# Autodesk Inventor assembly: CAMINHÃO BETONEIRA
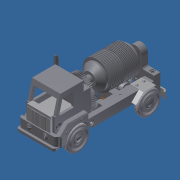
[picture p0: Inventor's stored thumbnail of the model, 180x180]
Saved by Autodesk Inventor 2012 SP2 (Build 160219200, 219)
## iProperties
Created: 2012-07-24
Part Number: CAMINHÃO BETONEIRA
Document SubType Name: Assembly
Designer: bruno.silveira
Author: bruno.silveira
## Documents named in this file (48)
- H:\CAD\BASSOTTI\Documents\DESENHOS.CAD-BRUNOBASSOTTI\DESENHOS-AUTODESK-INVENTOR\CAMINHÃO-BITONEIRA-(SENAI)\CAMINHÃO BETONEIRA.iam
- H:\CAD\BASSOTTI\Documents\DESENHOS.CAD-BRUNOBASSOTTI\DESENHOS-AUTODESK-INVENTOR\CAMINHÃO-BITONEIRA-(SENAI)\MOTOR(3).ipt
- H:\CAD\BASSOTTI\Documents\DESENHOS.CAD-BRUNOBASSOTTI\DESENHOS-AUTODESK-INVENTOR\CAMINHÃO-BITONEIRA-(SENAI)\LAT-CABINE-DIREITA(27).ipt
- H:\CAD\BASSOTTI\Documents\DESENHOS.CAD-BRUNOBASSOTTI\DESENHOS-AUTODESK-INVENTOR\CAMINHÃO-BITONEIRA-(SENAI)\LAT-CABINE-ESQUERDA(28).ipt
- H:\CAD\BASSOTTI\Documents\DESENHOS.CAD-BRUNOBASSOTTI\DESENHOS-AUTODESK-INVENTOR\CAMINHÃO-BITONEIRA-(SENAI)\ISO 2010 - M6x12.ipt
- H:\CAD\BASSOTTI\Documents\DESENHOS.CAD-BRUNOBASSOTTI\DESENHOS-AUTODESK-INVENTOR\CAMINHÃO-BITONEIRA-(SENAI)\PÁRA-LAMAS DIANTEIRO-DIR(1).ipt
- H:\CAD\BASSOTTI\Documents\DESENHOS.CAD-BRUNOBASSOTTI\DESENHOS-AUTODESK-INVENTOR\CAMINHÃO-BITONEIRA-(SENAI)\PÁRA-LAMAS DIANTEIRO-ESQ(1).ipt
- H:\CAD\BASSOTTI\Documents\DESENHOS.CAD-BRUNOBASSOTTI\DESENHOS-AUTODESK-INVENTOR\CAMINHÃO-BITONEIRA-(SENAI)\DIN 661 - A 3 x 16 x 11.ipt
- H:\CAD\BASSOTTI\Documents\DESENHOS.CAD-BRUNOBASSOTTI\DESENHOS-AUTODESK-INVENTOR\CAMINHÃO-BITONEIRA-(SENAI)\TRASEIRA DA CABINE(12).ipt
- H:\CAD\BASSOTTI\Documents\DESENHOS.CAD-BRUNOBASSOTTI\DESENHOS-AUTODESK-INVENTOR\CAMINHÃO-BITONEIRA-(SENAI)\TETO DA CABINE(15).ipt
- H:\CAD\BASSOTTI\Documents\DESENHOS.CAD-BRUNOBASSOTTI\DESENHOS-AUTODESK-INVENTOR\CAMINHÃO-BITONEIRA-(SENAI)\ISO 2010 - M6x10.ipt
- H:\CAD\BASSOTTI\Documents\DESENHOS.CAD-BRUNOBASSOTTI\DESENHOS-AUTODESK-INVENTOR\CAMINHÃO-BITONEIRA-(SENAI)\PÁRA-CHOQUE DIANTEIRO(4).ipt
- H:\CAD\BASSOTTI\Documents\DESENHOS.CAD-BRUNOBASSOTTI\DESENHOS-AUTODESK-INVENTOR\CAMINHÃO-BITONEIRA-(SENAI)\ASSOALHO(8).ipt
- H:\CAD\BASSOTTI\Documents\DESENHOS.CAD-BRUNOBASSOTTI\DESENHOS-AUTODESK-INVENTOR\CAMINHÃO-BITONEIRA-(SENAI)\MANCAL DO EIXO DIANTEIRO(7).ipt
- H:\CAD\BASSOTTI\Documents\DESENHOS.CAD-BRUNOBASSOTTI\DESENHOS-AUTODESK-INVENTOR\CAMINHÃO-BITONEIRA-(SENAI)\ISO 4762 - M6 x 16ISO.ipt
- H:\CAD\BASSOTTI\Documents\DESENHOS.CAD-BRUNOBASSOTTI\DESENHOS-AUTODESK-INVENTOR\CAMINHÃO-BITONEIRA-(SENAI)\EIXO DIANTEIRO(34).ipt
- H:\CAD\BASSOTTI\Documents\DESENHOS.CAD-BRUNOBASSOTTI\DESENHOS-AUTODESK-INVENTOR\CAMINHÃO-BITONEIRA-(SENAI)\RODA(33).ipt
- H:\CAD\BASSOTTI\Documents\DESENHOS.CAD-BRUNOBASSOTTI\DESENHOS-AUTODESK-INVENTOR\CAMINHÃO-BITONEIRA-(SENAI)\ARRUELA ESPECIAL DAS RODAS(31).ipt
- H:\CAD\BASSOTTI\Documents\DESENHOS.CAD-BRUNOBASSOTTI\DESENHOS-AUTODESK-INVENTOR\CAMINHÃO-BITONEIRA-(SENAI)\DIN 913 - M6 x 8.ipt
- H:\CAD\BASSOTTI\Documents\DESENHOS.CAD-BRUNOBASSOTTI\DESENHOS-AUTODESK-INVENTOR\CAMINHÃO-BITONEIRA-(SENAI)\PLACA COM FUROS COORDENADOS(13).ipt
- H:\CAD\BASSOTTI\Documents\DESENHOS.CAD-BRUNOBASSOTTI\DESENHOS-AUTODESK-INVENTOR\CAMINHÃO-BITONEIRA-(SENAI)\CHASSI DIREITO(58).ipt
- H:\CAD\BASSOTTI\Documents\DESENHOS.CAD-BRUNOBASSOTTI\DESENHOS-AUTODESK-INVENTOR\CAMINHÃO-BITONEIRA-(SENAI)\CHASSI ESQUERDO(37).ipt
- H:\CAD\BASSOTTI\Documents\DESENHOS.CAD-BRUNOBASSOTTI\DESENHOS-AUTODESK-INVENTOR\CAMINHÃO-BITONEIRA-(SENAI)\PÁRA-LAMA TRASEIRO(50).ipt
- H:\CAD\BASSOTTI\Documents\DESENHOS.CAD-BRUNOBASSOTTI\DESENHOS-AUTODESK-INVENTOR\CAMINHÃO-BITONEIRA-(SENAI)\Rivet GB_T 827-1986-3 X 12.ipt
- H:\CAD\BASSOTTI\Documents\DESENHOS.CAD-BRUNOBASSOTTI\DESENHOS-AUTODESK-INVENTOR\CAMINHÃO-BITONEIRA-(SENAI)\SUPORTE DO EIXO TRASEIRO(51).ipt
- H:\CAD\BASSOTTI\Documents\DESENHOS.CAD-BRUNOBASSOTTI\DESENHOS-AUTODESK-INVENTOR\CAMINHÃO-BITONEIRA-(SENAI)\EIXO EXCÊNTRICO(53).ipt
- H:\CAD\BASSOTTI\Documents\DESENHOS.CAD-BRUNOBASSOTTI\DESENHOS-AUTODESK-INVENTOR\CAMINHÃO-BITONEIRA-(SENAI)\EIXO DAS ENGRENAGENS(11).ipt
- H:\CAD\BASSOTTI\Documents\DESENHOS.CAD-BRUNOBASSOTTI\DESENHOS-AUTODESK-INVENTOR\CAMINHÃO-BITONEIRA-(SENAI)\BUCHA DA PLACA(38).ipt
- H:\CAD\BASSOTTI\Documents\DESENHOS.CAD-BRUNOBASSOTTI\DESENHOS-AUTODESK-INVENTOR\CAMINHÃO-BITONEIRA-(SENAI)\ENGR.RETA MOTORA(18)\ENGR.RETA MOTORA(18).ipt
- H:\CAD\BASSOTTI\Documents\DESENHOS.CAD-BRUNOBASSOTTI\DESENHOS-AUTODESK-INVENTOR\CAMINHÃO-BITONEIRA-(SENAI)\ENGR.HELICOIDAL MOVIDA(59)\ENGR.HELICOIDAL MOVIDA(59).iam
- H:\CAD\BASSOTTI\Documents\DESENHOS.CAD-BRUNOBASSOTTI\DESENHOS-AUTODESK-INVENTOR\CAMINHÃO-BITONEIRA-(SENAI)\ISO 2339 - A - 4 x 24ISO.ipt
- H:\CAD\BASSOTTI\Documents\DESENHOS.CAD-BRUNOBASSOTTI\DESENHOS-AUTODESK-INVENTOR\CAMINHÃO-BITONEIRA-(SENAI)\MANCAL DA BETONEIRA(26).ipt
- H:\CAD\BASSOTTI\Documents\DESENHOS.CAD-BRUNOBASSOTTI\DESENHOS-AUTODESK-INVENTOR\CAMINHÃO-BITONEIRA-(SENAI)\MANCAL DO EIXO CARDAN(57).ipt
- H:\CAD\BASSOTTI\Documents\DESENHOS.CAD-BRUNOBASSOTTI\DESENHOS-AUTODESK-INVENTOR\CAMINHÃO-BITONEIRA-(SENAI)\ISO 4762 - M6 x 12ISO.ipt
- H:\CAD\BASSOTTI\Documents\DESENHOS.CAD-BRUNOBASSOTTI\DESENHOS-AUTODESK-INVENTOR\CAMINHÃO-BITONEIRA-(SENAI)\ENGR.HELICOIDAL MOTORA(20)\ENGR.HELICOIDAL MOTORA(20).ipt
- H:\CAD\BASSOTTI\Documents\DESENHOS.CAD-BRUNOBASSOTTI\DESENHOS-AUTODESK-INVENTOR\CAMINHÃO-BITONEIRA-(SENAI)\BUCHA DO MANCAL(41).ipt
- H:\CAD\BASSOTTI\Documents\DESENHOS.CAD-BRUNOBASSOTTI\DESENHOS-AUTODESK-INVENTOR\CAMINHÃO-BITONEIRA-(SENAI)\ENGR.RETA MOVIDA(17)\ENGR.RETA MOVIDA(17).ipt
- H:\CAD\BASSOTTI\Documents\DESENHOS.CAD-BRUNOBASSOTTI\DESENHOS-AUTODESK-INVENTOR\CAMINHÃO-BITONEIRA-(SENAI)\EIXO DA BETONEIRA(21).ipt
- H:\CAD\BASSOTTI\Documents\DESENHOS.CAD-BRUNOBASSOTTI\DESENHOS-AUTODESK-INVENTOR\CAMINHÃO-BITONEIRA-(SENAI)\ISO 2339 - A - 3 x 16ISO.ipt
- H:\CAD\BASSOTTI\Documents\DESENHOS.CAD-BRUNOBASSOTTI\DESENHOS-AUTODESK-INVENTOR\CAMINHÃO-BITONEIRA-(SENAI)\PÁRA-CHOQUE TRASEIRO\PÁRA-CHOQUE TRASEIRO.iam
- H:\CAD\BASSOTTI\Documents\DESENHOS.CAD-BRUNOBASSOTTI\DESENHOS-AUTODESK-INVENTOR\CAMINHÃO-BITONEIRA-(SENAI)\PINO ROSCADO(25).ipt
- H:\CAD\BASSOTTI\Documents\DESENHOS.CAD-BRUNOBASSOTTI\DESENHOS-AUTODESK-INVENTOR\CAMINHÃO-BITONEIRA-(SENAI)\COROA(43) - PINHÃO(54)\COROA(43) - PINHÃO(54).iam
- H:\CAD\BASSOTTI\Documents\DESENHOS.CAD-BRUNOBASSOTTI\DESENHOS-AUTODESK-INVENTOR\CAMINHÃO-BITONEIRA-(SENAI)\LUVA COM ROSCA TRAPEZOIDAL(22).ipt
- H:\CAD\BASSOTTI\Documents\DESENHOS.CAD-BRUNOBASSOTTI\DESENHOS-AUTODESK-INVENTOR\CAMINHÃO-BITONEIRA-(SENAI)\LUVA CÔNICA COM ROSCA MULTIPLA(23).ipt
- H:\CAD\BASSOTTI\Documents\DESENHOS.CAD-BRUNOBASSOTTI\DESENHOS-AUTODESK-INVENTOR\CAMINHÃO-BITONEIRA-(SENAI)\LUVA(24).ipt
- H:\CAD\BASSOTTI\Documents\DESENHOS.CAD-BRUNOBASSOTTI\DESENHOS-AUTODESK-INVENTOR\CAMINHÃO-BITONEIRA-(SENAI)\ESCAPAMENTO(16).ipt
- H:\CAD\BASSOTTI\Documents\DESENHOS.CAD-BRUNOBASSOTTI\DESENHOS-AUTODESK-INVENTOR\CAMINHÃO-BITONEIRA-(SENAI)\ISO 2010 - M6x16.ipt
- H:\CAD\BASSOTTI\Documents\DESENHOS.CAD-BRUNOBASSOTTI\DESENHOS-AUTODESK-INVENTOR\CAMINHÃO-BITONEIRA-(SENAI)\ISO 2339 - A - 3 x 20ISO.ipt
## Components (87 placed, 46 different names)
1. MOTOR(3):1 — Mate:1, Mate:2, Flush:1, Mate:3, Mate:4, Mate:5, Mate:6, Mate:7, Mate:8, Mate:35, Mate:36, Mate:37, Mate:40, Mate:41, Mate:42, Mate:46, Mate:47
2. LAT-CABINE-DIREITA(27):1 — Mate:3, Mate:4, Mate:5, Mate:9, Tangent:1, Mate:10, Tangent:2, Mate:13, Mate:14, Mate:15, Mate:27, Flush:3
3. LAT-CABINE-ESQUERDA(28):1 — Mate:6, Mate:7, Mate:8, Mate:11, Tangent:3, Mate:12, Tangent:4, Mate:16, Mate:17, Mate:18, Mate:28, Flush:2
4. ISO 2010 - M6x12:1 — Mate:9, Tangent:1
5. ISO 2010 - M6x12:2 — Mate:10, Tangent:2
6. ISO 2010 - M6x12:3 — Mate:11, Tangent:3
7. ISO 2010 - M6x12:4 — Mate:12, Tangent:4
8. PÁRA-LAMAS DIANTEIRO-DIR(1):1 — Mate:16, Mate:17, Mate:18, Mate:23, Mate:24, Mate:25, Mate:26
9. PÁRA-LAMAS DIANTEIRO-ESQ(1):1 — Mate:13, Mate:14, Mate:15, Mate:19, Mate:20, Mate:21, Mate:22, Mate:70
10. DIN 661 - A 3 x 16 x 11:1 — Mate:19, Mate:20
11. DIN 661 - A 3 x 16 x 11:2 — Mate:21, Mate:22
12. DIN 661 - A 3 x 16 x 11:3 — Mate:23, Mate:24
13. DIN 661 - A 3 x 16 x 11:4 — Mate:25, Mate:26
14. TRASEIRA DA CABINE(12):1 — Mate:29, Mate:30, Flush:3, Mate:31, Mate:32, Mate:33, Mate:34, Tangent:5, Tangent:6, Tangent:7, Tangent:8, Mate:65, Mate:66, Mate:67, Mate:171, Mate:172, Tangent:22, Tangent:23
15. TETO DA CABINE(15):1 — Mate:27, Mate:28, Flush:2, Mate:29, Mate:30, Angle:4
16. ISO 2010 - M6x10:1 — Mate:31, Tangent:7
17. ISO 2010 - M6x10:2 — Mate:32, Tangent:8
18. ISO 2010 - M6x10:3 — Mate:34, Tangent:6
19. ISO 2010 - M6x10:4 — Mate:33, Tangent:5
20. PÁRA-CHOQUE DIANTEIRO(4):1 — Mate:35, Mate:36, Mate:37, Mate:38, Mate:39, Tangent:9, Tangent:10
21. ISO 2010 - M6x12:5 — Mate:38, Tangent:10
22. ISO 2010 - M6x12:6 — Mate:39, Tangent:9
23. ASSOALHO(8):1 — Mate:40, Mate:41, Mate:42, Mate:43, Mate:44, Mate:45, Tangent:11, Tangent:12, Tangent:13, Mate:48
24. ISO 2010 - M6x10:5 — Mate:43, Tangent:11
25. ISO 2010 - M6x10:6 — Mate:44, Tangent:13
26. ISO 2010 - M6x10:7 — Mate:45, Tangent:12
27. MANCAL DO EIXO DIANTEIRO(7):1 — Mate:46, Mate:47, Mate:48, Mate:49, Mate:50, Mate:51, Mate:56, Mate:57
28. ISO 4762 - M6 x 16ISO:1 — Mate:49, Mate:50
29. EIXO DIANTEIRO(34):1 — Mate:51, Mate:52, Mate:53, Mate:54, Mate:55, Mate:56, Mate:58
30. RODA(33):1 — Mate:52, Mate:55, Mate:59, Mate:60
31. RODA(33):2 — Mate:53, Mate:54, Mate:61, Mate:62
32. ARRUELA ESPECIAL DAS RODAS(31):1 — Mate:59, Mate:60, Mate:63, Tangent:14
33. ARRUELA ESPECIAL DAS RODAS(31):2 — Mate:61, Mate:62, Mate:64, Tangent:15
34. DIN 913 - M6 x 6:1 — Mate:57, Mate:58
35. ISO 2010 - M6x12:7 — Mate:63, Tangent:14
36. ISO 2010 - M6x12:8 — Mate:64, Tangent:15
37. PLACA COM FUROS COORDENADOS(13):1 — Mate:65, Mate:66, Mate:67, Mate:68, Mate:69, Mate:71, Mate:73, Mate:74, Mate:75, Mate:112, Mate:113, Mate:114, Mate:115, Mate:116, Mate:117, Mate:132, Mate:133, Mate:134, Mate:169
38. CHASSI DIREITO(58):1 — Mate:68, Mate:69, Mate:70, Mate:72, Mate:81, Mate:82, Mate:83, Mate:88, Mate:89, Mate:95, Mate:96, Mate:97, Mate:125, Mate:127, Mate:129, Mate:140, Mate:141, Mate:154
39. CHASSI ESQUERDO(37):1 — Mate:73, Mate:74, Mate:75, Mate:76, Mate:77, Mate:78, Mate:79, Mate:80, Mate:84, Mate:85, Mate:92, Mate:93, Mate:94, Mate:126, Mate:130, Mate:131, Mate:142, Mate:155, Mate:170
40. ISO 4762 - M6 x 16ISO:2 — Mate:71, Mate:72
41. ISO 4762 - M6 x 16ISO:3 — Mate:76, Mate:77
42. PÁRA-LAMA TRASEIRO(50):1 — Mate:78, Mate:79, Mate:80, Mate:86, Mate:87
43. PÁRA-LAMA TRASEIRO(50):2 — Mate:81, Mate:82, Mate:83, Mate:90, Mate:91
44. Rivet GB_T 827-1986-3 X 12:1 — Mate:85, Mate:86
45. Rivet GB_T 827-1986-3 X 12:2 — Mate:84, Mate:87
46. Rivet GB_T 827-1986-3 X 12:3 — Mate:89, Mate:90
47. Rivet GB_T 827-1986-3 X 12:4 — Mate:88, Mate:91
48. SUPORTE DO EIXO TRASEIRO(51):1 — Mate:92, Mate:93, Mate:94, Mate:98, Angle:1
49. SUPORTE DO EIXO TRASEIRO(51):2 — Mate:95, Mate:96, Mate:97, Mate:99
50. EIXO EXCÊNTRICO(53):1 — Mate:98, Mate:99, Mate:100, Mate:101, Mate:102, Mate:103, Mate:104, Mate:105, Angle:7, FUNCIONAMENTO
51. RODA(33):3 — Mate:100, Mate:101, Mate:104, Mate:106, Mate:107
52. RODA(33):4 — Mate:102, Mate:103, Mate:105, Mate:108, Mate:109
53. ARRUELA ESPECIAL DAS RODAS(31):3 — Mate:106, Mate:107, Mate:110, Tangent:16
54. ARRUELA ESPECIAL DAS RODAS(31):4 — Mate:108, Mate:109, Mate:111, Tangent:17
55. ISO 2010 - M6x12:9 — Mate:110, Tangent:16
56. ISO 2010 - M6x12:10 — Mate:111, Tangent:17
57. EIXO DAS ENGRENAGENS(11):1 — Mate:112, Mate:113, Mate:118, Mate:123
58. BUCHA DA PLACA(38):1 — Mate:115, Mate:117, Mate:119
59. BUCHA DA PLACA(38):2 — Mate:114, Mate:116, Mate:138, Mate:139
60. ENGR.RETA MOTORA(18):1 — Mate:118, Mate:119, Mate:120, Mate:121, Mate:122
61. ENGR.HELICOIDAL MOVIDA(59):1 [sub-assembly] — Mate:120, Mate:121, Mate:122, Mate:123, Mate:124, Tangent:18, Rotation:1, Rotation:2
62. ISO 2339 - A - 3 x 16ISO:1 — Mate:124, Tangent:18
63. MANCAL DA BETONEIRA(26):1 — Mate:140, Mate:141, Mate:142, Mate:147, Mate:148, Mate:149, Mate:150, Mate:151, Mate:152, Mate:153
64. MANCAL DO EIXO CARDAN(57):1 — Mate:125, Mate:126, Mate:127, Mate:128, Mate:135, Mate:136, Mate:161
65. ISO 4762 - M6 x 12ISO:1 — Mate:128, Mate:129
66. ISO 4762 - M6 x 12ISO:2 — Mate:130, Mate:131
67. ENGR.HELICOIDAL MOTORA(20):1 — Mate:132, Mate:137, Mate:160, Mate:162, Rotation:1
68. BUCHA DO MANCAL(41):1 — Mate:133, Mate:134, Mate:137
69. BUCHA DO MANCAL(41):2 — Mate:135, Mate:136
70. ENGR.RETA MOVIDA(17):1 — Mate:138, Mate:139, Mate:143, Mate:144, Mate:145, Rotation:2
71. EIXO DA BETONEIRA(21):1 — Mate:143, Mate:144, Mate:145, Mate:146, Tangent:19, Mate:159, Mate:163, Mate:164, Mate:165, Mate:167, Angle:5, Angle:6
72. ISO 2339 - A - 3 x 16ISO:2 — Mate:146, Tangent:19
73. BUCHA DA PLACA(38):3 — Mate:147, Mate:148, Mate:158
74. ISO 4762 - M6 x 12ISO:3 — Mate:149, Mate:152
75. ISO 4762 - M6 x 12ISO:4 — Mate:150, Mate:151
76. PÁRA-CHOQUE TRASEIRO:1 [sub-assembly] — Mate:153, Mate:154, Mate:155, Mate:156, Mate:157, Tangent:20, Tangent:21
77. ISO 2010 - M6x10:8 — Mate:156, Tangent:21
78. ISO 2010 - M6x10:9 — Mate:157, Tangent:20
79. PINO ROSCADO(25):1 — Mate:158, Mate:159
80. COROA(43) - PINHÃO(54):1 [sub-assembly] — Mate:160, Mate:161, Angle:1, Mate:162, Angle:7, Mate:173, Tangent:24
81. LUVA COM ROSCA TRAPEZOIDAL(22):1 — Mate:164, Mate:165, Mate:166, Angle:5
82. LUVA CÔNICA COM ROSCA MULTIPLA(23):1 — Mate:163, Mate:166, Mate:168, Angle:6
83. LUVA(24):1 — Mate:167, Mate:168
84. ESCAPAMENTO(16):1 — Mate:169, Mate:170, Angle:4
85. ISO 2010 - M6x16:1 — Mate:172, Tangent:22
86. ISO 2010 - M6x16:2 — Mate:171, Tangent:23
87. ISO 2339 - A - 3 x 20ISO:1 — Mate:173, Tangent:24
## Relationships (208: Mate 173, Tangent 24, Angle 6, Flush 3, RelateRotation 2)
- Mate:1: MOTOR(3):1
- Mate:2: MOTOR(3):1
- Flush:1: MOTOR(3):1
- Mate:3: MOTOR(3):1 ↔ LAT-CABINE-DIREITA(27):1
- Mate:4: MOTOR(3):1 ↔ LAT-CABINE-DIREITA(27):1
- Mate:5: MOTOR(3):1 ↔ LAT-CABINE-DIREITA(27):1
- Mate:6: MOTOR(3):1 ↔ LAT-CABINE-ESQUERDA(28):1
- Mate:7: MOTOR(3):1 ↔ LAT-CABINE-ESQUERDA(28):1
- Mate:8: MOTOR(3):1 ↔ LAT-CABINE-ESQUERDA(28):1
- Mate:9: LAT-CABINE-DIREITA(27):1 ↔ ISO 2010 - M6x12:1
- Tangent:1: LAT-CABINE-DIREITA(27):1 ↔ ISO 2010 - M6x12:1
- Mate:10: LAT-CABINE-DIREITA(27):1 ↔ ISO 2010 - M6x12:2
- Tangent:2: LAT-CABINE-DIREITA(27):1 ↔ ISO 2010 - M6x12:2
- Mate:11: LAT-CABINE-ESQUERDA(28):1 ↔ ISO 2010 - M6x12:3
- Tangent:3: LAT-CABINE-ESQUERDA(28):1 ↔ ISO 2010 - M6x12:3
- Mate:12: LAT-CABINE-ESQUERDA(28):1 ↔ ISO 2010 - M6x12:4
- Tangent:4: LAT-CABINE-ESQUERDA(28):1 ↔ ISO 2010 - M6x12:4
- Mate:13: LAT-CABINE-DIREITA(27):1 ↔ PÁRA-LAMAS DIANTEIRO-ESQ(1):1
- Mate:14: LAT-CABINE-DIREITA(27):1 ↔ PÁRA-LAMAS DIANTEIRO-ESQ(1):1
- Mate:15: LAT-CABINE-DIREITA(27):1 ↔ PÁRA-LAMAS DIANTEIRO-ESQ(1):1
- Mate:16: LAT-CABINE-ESQUERDA(28):1 ↔ PÁRA-LAMAS DIANTEIRO-DIR(1):1
- Mate:17: LAT-CABINE-ESQUERDA(28):1 ↔ PÁRA-LAMAS DIANTEIRO-DIR(1):1
- Mate:18: LAT-CABINE-ESQUERDA(28):1 ↔ PÁRA-LAMAS DIANTEIRO-DIR(1):1
- Mate:19: PÁRA-LAMAS DIANTEIRO-ESQ(1):1 ↔ DIN 661 - A 3 x 16 x 11:1
- Mate:20: PÁRA-LAMAS DIANTEIRO-ESQ(1):1 ↔ DIN 661 - A 3 x 16 x 11:1
- Mate:21: PÁRA-LAMAS DIANTEIRO-ESQ(1):1 ↔ DIN 661 - A 3 x 16 x 11:2
- Mate:22: PÁRA-LAMAS DIANTEIRO-ESQ(1):1 ↔ DIN 661 - A 3 x 16 x 11:2
- Mate:23: PÁRA-LAMAS DIANTEIRO-DIR(1):1 ↔ DIN 661 - A 3 x 16 x 11:3
- Mate:24: PÁRA-LAMAS DIANTEIRO-DIR(1):1 ↔ DIN 661 - A 3 x 16 x 11:3
- Mate:25: PÁRA-LAMAS DIANTEIRO-DIR(1):1 ↔ DIN 661 - A 3 x 16 x 11:4
- Mate:26: PÁRA-LAMAS DIANTEIRO-DIR(1):1 ↔ DIN 661 - A 3 x 16 x 11:4
- Mate:27: LAT-CABINE-DIREITA(27):1 ↔ TETO DA CABINE(15):1
- Mate:28: LAT-CABINE-ESQUERDA(28):1 ↔ TETO DA CABINE(15):1
- Flush:2: LAT-CABINE-ESQUERDA(28):1 ↔ TETO DA CABINE(15):1
- Mate:29: TRASEIRA DA CABINE(12):1 ↔ TETO DA CABINE(15):1
- Mate:30: TRASEIRA DA CABINE(12):1 ↔ TETO DA CABINE(15):1
- Flush:3: LAT-CABINE-DIREITA(27):1 ↔ TRASEIRA DA CABINE(12):1
- Mate:31: TRASEIRA DA CABINE(12):1 ↔ ISO 2010 - M6x10:1
- Mate:32: TRASEIRA DA CABINE(12):1 ↔ ISO 2010 - M6x10:2
- Mate:33: TRASEIRA DA CABINE(12):1 ↔ ISO 2010 - M6x10:4
- Mate:34: TRASEIRA DA CABINE(12):1 ↔ ISO 2010 - M6x10:3
- Tangent:5: TRASEIRA DA CABINE(12):1 ↔ ISO 2010 - M6x10:4
- Tangent:6: TRASEIRA DA CABINE(12):1 ↔ ISO 2010 - M6x10:3
- Tangent:7: TRASEIRA DA CABINE(12):1 ↔ ISO 2010 - M6x10:1
- Tangent:8: TRASEIRA DA CABINE(12):1 ↔ ISO 2010 - M6x10:2
- Mate:35: MOTOR(3):1 ↔ PÁRA-CHOQUE DIANTEIRO(4):1
- Mate:36: MOTOR(3):1 ↔ PÁRA-CHOQUE DIANTEIRO(4):1
- Mate:37: MOTOR(3):1 ↔ PÁRA-CHOQUE DIANTEIRO(4):1
- Mate:38: PÁRA-CHOQUE DIANTEIRO(4):1 ↔ ISO 2010 - M6x12:5
- Mate:39: PÁRA-CHOQUE DIANTEIRO(4):1 ↔ ISO 2010 - M6x12:6
- Tangent:9: PÁRA-CHOQUE DIANTEIRO(4):1 ↔ ISO 2010 - M6x12:6
- Tangent:10: PÁRA-CHOQUE DIANTEIRO(4):1 ↔ ISO 2010 - M6x12:5
- Mate:40: MOTOR(3):1 ↔ ASSOALHO(8):1
- Mate:41: MOTOR(3):1 ↔ ASSOALHO(8):1
- Mate:42: MOTOR(3):1 ↔ ASSOALHO(8):1
- Mate:43: ASSOALHO(8):1 ↔ ISO 2010 - M6x10:5
- Mate:44: ASSOALHO(8):1 ↔ ISO 2010 - M6x10:6
- Mate:45: ASSOALHO(8):1 ↔ ISO 2010 - M6x10:7
- Tangent:11: ASSOALHO(8):1 ↔ ISO 2010 - M6x10:5
- Tangent:12: ASSOALHO(8):1 ↔ ISO 2010 - M6x10:7
- Tangent:13: ASSOALHO(8):1 ↔ ISO 2010 - M6x10:6
- Mate:46: MOTOR(3):1 ↔ MANCAL DO EIXO DIANTEIRO(7):1
- Mate:47: MOTOR(3):1 ↔ MANCAL DO EIXO DIANTEIRO(7):1
- Mate:48: ASSOALHO(8):1 ↔ MANCAL DO EIXO DIANTEIRO(7):1
- Mate:49: MANCAL DO EIXO DIANTEIRO(7):1 ↔ ISO 4762 - M6 x 16ISO:1
- Mate:50: MANCAL DO EIXO DIANTEIRO(7):1 ↔ ISO 4762 - M6 x 16ISO:1
- Mate:51: MANCAL DO EIXO DIANTEIRO(7):1 ↔ EIXO DIANTEIRO(34):1
- Mate:52: EIXO DIANTEIRO(34):1 ↔ RODA(33):1
- Mate:53: EIXO DIANTEIRO(34):1 ↔ RODA(33):2
- Mate:54: EIXO DIANTEIRO(34):1 ↔ RODA(33):2
- Mate:55: EIXO DIANTEIRO(34):1 ↔ RODA(33):1
- Mate:56: MANCAL DO EIXO DIANTEIRO(7):1 ↔ EIXO DIANTEIRO(34):1
- Mate:57: MANCAL DO EIXO DIANTEIRO(7):1 ↔ DIN 913 - M6 x 6:1
- Mate:58: EIXO DIANTEIRO(34):1 ↔ DIN 913 - M6 x 6:1
- Mate:59: RODA(33):1 ↔ ARRUELA ESPECIAL DAS RODAS(31):1
- Mate:60: RODA(33):1 ↔ ARRUELA ESPECIAL DAS RODAS(31):1
- Mate:61: RODA(33):2 ↔ ARRUELA ESPECIAL DAS RODAS(31):2
- Mate:62: RODA(33):2 ↔ ARRUELA ESPECIAL DAS RODAS(31):2
- Mate:63: ARRUELA ESPECIAL DAS RODAS(31):1 ↔ ISO 2010 - M6x12:7
- Tangent:14: ARRUELA ESPECIAL DAS RODAS(31):1 ↔ ISO 2010 - M6x12:7
- Mate:64: ARRUELA ESPECIAL DAS RODAS(31):2 ↔ ISO 2010 - M6x12:8
- Tangent:15: ARRUELA ESPECIAL DAS RODAS(31):2 ↔ ISO 2010 - M6x12:8
- Mate:65: TRASEIRA DA CABINE(12):1 ↔ PLACA COM FUROS COORDENADOS(13):1
- Mate:66: TRASEIRA DA CABINE(12):1 ↔ PLACA COM FUROS COORDENADOS(13):1
- Mate:67: TRASEIRA DA CABINE(12):1 ↔ PLACA COM FUROS COORDENADOS(13):1
- Mate:68: PLACA COM FUROS COORDENADOS(13):1 ↔ CHASSI DIREITO(58):1
- Mate:69: PLACA COM FUROS COORDENADOS(13):1 ↔ CHASSI DIREITO(58):1
- Mate:70: PÁRA-LAMAS DIANTEIRO-ESQ(1):1 ↔ CHASSI DIREITO(58):1
- Mate:71: PLACA COM FUROS COORDENADOS(13):1 ↔ ISO 4762 - M6 x 16ISO:2
- Mate:72: CHASSI DIREITO(58):1 ↔ ISO 4762 - M6 x 16ISO:2
- Mate:73: PLACA COM FUROS COORDENADOS(13):1 ↔ CHASSI ESQUERDO(37):1
- Mate:74: PLACA COM FUROS COORDENADOS(13):1 ↔ CHASSI ESQUERDO(37):1
- Mate:75: PLACA COM FUROS COORDENADOS(13):1 ↔ CHASSI ESQUERDO(37):1
- Mate:76: CHASSI ESQUERDO(37):1 ↔ ISO 4762 - M6 x 16ISO:3
- Mate:77: CHASSI ESQUERDO(37):1 ↔ ISO 4762 - M6 x 16ISO:3
- Mate:78: CHASSI ESQUERDO(37):1 ↔ PÁRA-LAMA TRASEIRO(50):1
- Mate:79: CHASSI ESQUERDO(37):1 ↔ PÁRA-LAMA TRASEIRO(50):1
- Mate:80: CHASSI ESQUERDO(37):1 ↔ PÁRA-LAMA TRASEIRO(50):1
- Mate:81: CHASSI DIREITO(58):1 ↔ PÁRA-LAMA TRASEIRO(50):2
- Mate:82: CHASSI DIREITO(58):1 ↔ PÁRA-LAMA TRASEIRO(50):2
- Mate:83: CHASSI DIREITO(58):1 ↔ PÁRA-LAMA TRASEIRO(50):2
- Mate:84: CHASSI ESQUERDO(37):1 ↔ Rivet GB_T 827-1986-3 X 12:2
- Mate:85: CHASSI ESQUERDO(37):1 ↔ Rivet GB_T 827-1986-3 X 12:1
- Mate:86: PÁRA-LAMA TRASEIRO(50):1 ↔ Rivet GB_T 827-1986-3 X 12:1
- Mate:87: PÁRA-LAMA TRASEIRO(50):1 ↔ Rivet GB_T 827-1986-3 X 12:2
- Mate:88: CHASSI DIREITO(58):1 ↔ Rivet GB_T 827-1986-3 X 12:4
- Mate:89: CHASSI DIREITO(58):1 ↔ Rivet GB_T 827-1986-3 X 12:3
- Mate:90: PÁRA-LAMA TRASEIRO(50):2 ↔ Rivet GB_T 827-1986-3 X 12:3
- Mate:91: PÁRA-LAMA TRASEIRO(50):2 ↔ Rivet GB_T 827-1986-3 X 12:4
- Mate:92: CHASSI ESQUERDO(37):1 ↔ SUPORTE DO EIXO TRASEIRO(51):1
- Mate:93: CHASSI ESQUERDO(37):1 ↔ SUPORTE DO EIXO TRASEIRO(51):1
- Mate:94: CHASSI ESQUERDO(37):1 ↔ SUPORTE DO EIXO TRASEIRO(51):1
- Mate:95: CHASSI DIREITO(58):1 ↔ SUPORTE DO EIXO TRASEIRO(51):2
- Mate:96: CHASSI DIREITO(58):1 ↔ SUPORTE DO EIXO TRASEIRO(51):2
- Mate:97: CHASSI DIREITO(58):1 ↔ SUPORTE DO EIXO TRASEIRO(51):2
- Mate:98: SUPORTE DO EIXO TRASEIRO(51):1 ↔ EIXO EXCÊNTRICO(53):1
- Mate:99 (0.2 mm): SUPORTE DO EIXO TRASEIRO(51):2 ↔ EIXO EXCÊNTRICO(53):1
- Mate:100: EIXO EXCÊNTRICO(53):1 ↔ RODA(33):3
- Mate:101: EIXO EXCÊNTRICO(53):1 ↔ RODA(33):3
- Mate:102: EIXO EXCÊNTRICO(53):1 ↔ RODA(33):4
- Mate:103: EIXO EXCÊNTRICO(53):1 ↔ RODA(33):4
- Mate:104: EIXO EXCÊNTRICO(53):1 ↔ RODA(33):3
- Mate:105: EIXO EXCÊNTRICO(53):1 ↔ RODA(33):4
- Mate:106: RODA(33):3 ↔ ARRUELA ESPECIAL DAS RODAS(31):3
- Mate:107: RODA(33):3 ↔ ARRUELA ESPECIAL DAS RODAS(31):3
- Mate:108: RODA(33):4 ↔ ARRUELA ESPECIAL DAS RODAS(31):4
- Mate:109: RODA(33):4 ↔ ARRUELA ESPECIAL DAS RODAS(31):4
- Mate:110: ARRUELA ESPECIAL DAS RODAS(31):3 ↔ ISO 2010 - M6x12:9
- Tangent:16: ARRUELA ESPECIAL DAS RODAS(31):3 ↔ ISO 2010 - M6x12:9
- Mate:111: ARRUELA ESPECIAL DAS RODAS(31):4 ↔ ISO 2010 - M6x12:10
- Tangent:17: ARRUELA ESPECIAL DAS RODAS(31):4 ↔ ISO 2010 - M6x12:10
- Mate:112: PLACA COM FUROS COORDENADOS(13):1 ↔ EIXO DAS ENGRENAGENS(11):1
- Mate:113: PLACA COM FUROS COORDENADOS(13):1 ↔ EIXO DAS ENGRENAGENS(11):1
- Mate:114: PLACA COM FUROS COORDENADOS(13):1 ↔ BUCHA DA PLACA(38):2
- Mate:115: PLACA COM FUROS COORDENADOS(13):1 ↔ BUCHA DA PLACA(38):1
- Mate:116: PLACA COM FUROS COORDENADOS(13):1 ↔ BUCHA DA PLACA(38):2
- Mate:117: PLACA COM FUROS COORDENADOS(13):1 ↔ BUCHA DA PLACA(38):1
- Mate:118: EIXO DAS ENGRENAGENS(11):1 ↔ ENGR.RETA MOTORA(18):1
- Mate:119: BUCHA DA PLACA(38):1 ↔ ENGR.RETA MOTORA(18):1
- Mate:120: ENGR.RETA MOTORA(18):1 ↔ ENGR.HELICOIDAL MOVIDA(59):1
- Mate:121: ENGR.RETA MOTORA(18):1 ↔ ENGR.HELICOIDAL MOVIDA(59):1
- Mate:122: ENGR.RETA MOTORA(18):1 ↔ ENGR.HELICOIDAL MOVIDA(59):1
- Mate:123: EIXO DAS ENGRENAGENS(11):1 ↔ ENGR.HELICOIDAL MOVIDA(59):1
- Mate:124: ENGR.HELICOIDAL MOVIDA(59):1 ↔ ISO 2339 - A - 3 x 16ISO:1
- Tangent:18: ENGR.HELICOIDAL MOVIDA(59):1 ↔ ISO 2339 - A - 3 x 16ISO:1
- Mate:125: CHASSI DIREITO(58):1 ↔ MANCAL DO EIXO CARDAN(57):1
- Mate:126: CHASSI ESQUERDO(37):1 ↔ MANCAL DO EIXO CARDAN(57):1
- Mate:127: CHASSI DIREITO(58):1 ↔ MANCAL DO EIXO CARDAN(57):1
- Mate:128: MANCAL DO EIXO CARDAN(57):1 ↔ ISO 4762 - M6 x 12ISO:1
- Mate:129: CHASSI DIREITO(58):1 ↔ ISO 4762 - M6 x 12ISO:1
- Mate:130: CHASSI ESQUERDO(37):1 ↔ ISO 4762 - M6 x 12ISO:2
- Mate:131: CHASSI ESQUERDO(37):1 ↔ ISO 4762 - M6 x 12ISO:2
- Mate:132: PLACA COM FUROS COORDENADOS(13):1 ↔ ENGR.HELICOIDAL MOTORA(20):1
- Mate:133: PLACA COM FUROS COORDENADOS(13):1 ↔ BUCHA DO MANCAL(41):1
- Mate:134: PLACA COM FUROS COORDENADOS(13):1 ↔ BUCHA DO MANCAL(41):1
- Mate:135: MANCAL DO EIXO CARDAN(57):1 ↔ BUCHA DO MANCAL(41):2
- Mate:136: MANCAL DO EIXO CARDAN(57):1 ↔ BUCHA DO MANCAL(41):2
- Mate:137: ENGR.HELICOIDAL MOTORA(20):1 ↔ BUCHA DO MANCAL(41):1
- Mate:138: BUCHA DA PLACA(38):2 ↔ ENGR.RETA MOVIDA(17):1
- Mate:139: BUCHA DA PLACA(38):2 ↔ ENGR.RETA MOVIDA(17):1
- Mate:140: CHASSI DIREITO(58):1 ↔ MANCAL DA BETONEIRA(26):1
- Mate:141: CHASSI DIREITO(58):1 ↔ MANCAL DA BETONEIRA(26):1
- Mate:142: CHASSI ESQUERDO(37):1 ↔ MANCAL DA BETONEIRA(26):1
- Mate:143: ENGR.RETA MOVIDA(17):1 ↔ EIXO DA BETONEIRA(21):1
- Mate:144: ENGR.RETA MOVIDA(17):1 ↔ EIXO DA BETONEIRA(21):1
- Mate:145: ENGR.RETA MOVIDA(17):1 ↔ EIXO DA BETONEIRA(21):1
- Mate:146: EIXO DA BETONEIRA(21):1 ↔ ISO 2339 - A - 3 x 16ISO:2
- Tangent:19: EIXO DA BETONEIRA(21):1 ↔ ISO 2339 - A - 3 x 16ISO:2
- Mate:147: MANCAL DA BETONEIRA(26):1 ↔ BUCHA DA PLACA(38):3
- Mate:148: MANCAL DA BETONEIRA(26):1 ↔ BUCHA DA PLACA(38):3
- Mate:149: MANCAL DA BETONEIRA(26):1 ↔ ISO 4762 - M6 x 12ISO:3
- Mate:150: MANCAL DA BETONEIRA(26):1 ↔ ISO 4762 - M6 x 12ISO:4
- Mate:151: MANCAL DA BETONEIRA(26):1 ↔ ISO 4762 - M6 x 12ISO:4
- Mate:152: MANCAL DA BETONEIRA(26):1 ↔ ISO 4762 - M6 x 12ISO:3
- Mate:153: MANCAL DA BETONEIRA(26):1 ↔ PÁRA-CHOQUE TRASEIRO:1
- Mate:154: CHASSI DIREITO(58):1 ↔ PÁRA-CHOQUE TRASEIRO:1
- Mate:155: CHASSI ESQUERDO(37):1 ↔ PÁRA-CHOQUE TRASEIRO:1
- Mate:156: PÁRA-CHOQUE TRASEIRO:1 ↔ ISO 2010 - M6x10:8
- Mate:157: PÁRA-CHOQUE TRASEIRO:1 ↔ ISO 2010 - M6x10:9
- Tangent:20: PÁRA-CHOQUE TRASEIRO:1 ↔ ISO 2010 - M6x10:9
- Tangent:21: PÁRA-CHOQUE TRASEIRO:1 ↔ ISO 2010 - M6x10:8
- Mate:158: BUCHA DA PLACA(38):3 ↔ PINO ROSCADO(25):1
- Mate:159: EIXO DA BETONEIRA(21):1 ↔ PINO ROSCADO(25):1
- Mate:160: ENGR.HELICOIDAL MOTORA(20):1 ↔ COROA(43) - PINHÃO(54):1
- Mate:161: MANCAL DO EIXO CARDAN(57):1 ↔ COROA(43) - PINHÃO(54):1
- Angle:1 (0 deg): SUPORTE DO EIXO TRASEIRO(51):1 ↔ COROA(43) - PINHÃO(54):1
- Mate:162: ENGR.HELICOIDAL MOTORA(20):1 ↔ COROA(43) - PINHÃO(54):1
- Mate:163: EIXO DA BETONEIRA(21):1 ↔ LUVA CÔNICA COM ROSCA MULTIPLA(23):1
- Mate:164: EIXO DA BETONEIRA(21):1 ↔ LUVA COM ROSCA TRAPEZOIDAL(22):1
- Mate:165: EIXO DA BETONEIRA(21):1 ↔ LUVA COM ROSCA TRAPEZOIDAL(22):1
- Mate:166: LUVA COM ROSCA TRAPEZOIDAL(22):1 ↔ LUVA CÔNICA COM ROSCA MULTIPLA(23):1
- Mate:167: EIXO DA BETONEIRA(21):1 ↔ LUVA(24):1
- Mate:168: LUVA CÔNICA COM ROSCA MULTIPLA(23):1 ↔ LUVA(24):1
- Mate:169: PLACA COM FUROS COORDENADOS(13):1 ↔ ESCAPAMENTO(16):1
- Mate:170: CHASSI ESQUERDO(37):1 ↔ ESCAPAMENTO(16):1
- Angle:4 (180 deg): TETO DA CABINE(15):1 ↔ ESCAPAMENTO(16):1
- Mate:171: TRASEIRA DA CABINE(12):1 ↔ ISO 2010 - M6x16:2
- Mate:172: TRASEIRA DA CABINE(12):1 ↔ ISO 2010 - M6x16:1
- Tangent:22: TRASEIRA DA CABINE(12):1 ↔ ISO 2010 - M6x16:1
- Tangent:23: TRASEIRA DA CABINE(12):1 ↔ ISO 2010 - M6x16:2
- Angle:5 (0 deg): EIXO DA BETONEIRA(21):1 ↔ LUVA COM ROSCA TRAPEZOIDAL(22):1
- Angle:6 (0 deg): EIXO DA BETONEIRA(21):1 ↔ LUVA CÔNICA COM ROSCA MULTIPLA(23):1
- Angle:7 (0 deg): EIXO EXCÊNTRICO(53):1 ↔ COROA(43) - PINHÃO(54):1
- Mate:173: COROA(43) - PINHÃO(54):1 ↔ ISO 2339 - A - 3 x 20ISO:1
- Tangent:24: COROA(43) - PINHÃO(54):1 ↔ ISO 2339 - A - 3 x 20ISO:1
- Rotation:1 [RelateRotation] (1 ul): ENGR.HELICOIDAL MOVIDA(59):1 ↔ ENGR.HELICOIDAL MOTORA(20):1
- Rotation:2 [RelateRotation] (1 ul): ENGR.HELICOIDAL MOVIDA(59):1 ↔ ENGR.RETA MOVIDA(17):1
- FUNCIONAMENTO [Angle] (0 deg): EIXO EXCÊNTRICO(53):1
